# Autodesk Inventor assembly: FullyAssembled
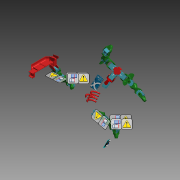
[picture p0: Inventor's stored thumbnail of the model, 180x180]
Saved by Autodesk Inventor 2015 (Build 190159000, 159)
## iProperties
Created: 2015-03-03
Part Number: FullyAssembled
Document SubType Name: Assembly
Designer: Henke
Author: Henke
## Documents named in this file (9)
- D:\Study_and_Projects\KTH\KEX i robotik\CAD\FullyAssembled.iam
- D:\Study_and_Projects\KTH\KEX i robotik\CAD\RearLegsWithHip.iam
- D:\Study_and_Projects\KTH\KEX i robotik\CAD\SpineConnector.ipt
- D:\Study_and_Projects\KTH\KEX i robotik\CAD\Servo with wheel.iam
- D:\Study_and_Projects\KTH\KEX i robotik\CAD\Arduino Mega 2560\Assembly1.iam
- D:\Study_and_Projects\KTH\KEX i robotik\CAD\DCDCStepDown\Imported Components\Step Down voltage regulator LM2596\Step Down voltage regulator LM2596.ipt
- D:\Study_and_Projects\KTH\KEX i robotik\CAD\RibBone.ipt
- D:\Study_and_Projects\KTH\KEX i robotik\CAD\Leg3DOF-Front.iam
- D:\Study_and_Projects\KTH\KEX i robotik\CAD\ChestConnector10Degrees.ipt
## Components (14 placed, 8 different names)
1. RearLegsWithHip:1 [sub-assembly] — Mate:2, Mate:3, Flush:1
2. SpineConnector:1 — Rotational:1, Rotational:2
3. Servo with wheel:1 [sub-assembly] — Rotational:2
4. Servo with wheel:2 [sub-assembly] — Mate:2, Mate:3, Flush:1, Rotational:1
5. Assembly1:1 [sub-assembly]
6. Step Down voltage regulator LM2596:1
7. RibBone:1
8. RibBone:2
9. RibBone:3
10. RibBone:4
11. RibBone:5
12. Leg3DOF-Front:1 [sub-assembly]
13. Leg3DOF-Front:2 [sub-assembly] — Mate:4, Mate:5
14. ChestConnector10Degrees:1 — Mate:4, Mate:5
## Relationships (7: Mate 4, RevoluteJoint 2, Flush 1)
- Mate:2: RearLegsWithHip:1 ↔ Servo with wheel:2
- Mate:3: RearLegsWithHip:1 ↔ Servo with wheel:2
- Flush:1: RearLegsWithHip:1 ↔ Servo with wheel:2
- Rotational:1 [RevoluteJoint]: SpineConnector:1 ↔ Servo with wheel:2
- Rotational:2 [RevoluteJoint]: SpineConnector:1 ↔ Servo with wheel:1
- Mate:4: Leg3DOF-Front:2 ↔ ChestConnector10Degrees:1
- Mate:5: Leg3DOF-Front:2 ↔ ChestConnector10Degrees:1
